# Autodesk Inventor assembly: Chassis Assembly
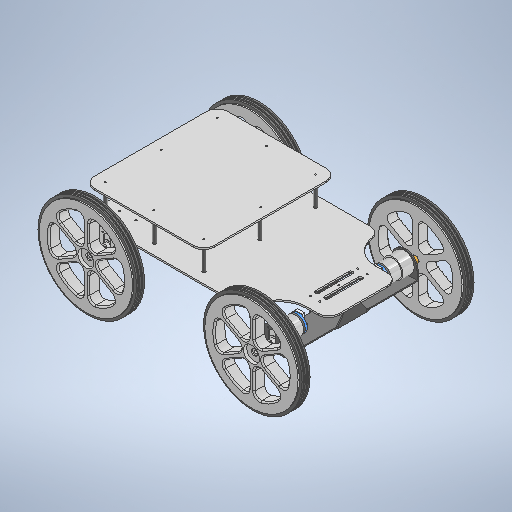
[picture p0: Inventor's stored thumbnail of the model, 512x512]
Saved by Autodesk Inventor 2025.2 (Build 292293000, 293)
## iProperties
Created: 2025-01-16
Part Number: Chassis Assembly
Document SubType Name: Assembly
Designer: Matt Tidd
Author: Matt Tidd
## Documents named in this file (6)
- C:\Users\mtidd2\Desktop\H2A\CAD\Chassis_Design\Chassis Assembly.iam
- C:\Users\mtidd2\Desktop\H2A\CAD\Motors_and_Wheels\Pendulum Suspension\Pendulum Suspension Assembly.iam
- C:\Users\mtidd2\Desktop\H2A\CAD\Chassis_Design\Chassis Bottom Plate.ipt
- C:\Users\mtidd2\Desktop\H2A\CAD\Motors_and_Wheels\Wheel Assembly\Motor Wheel Assembly.iam
- C:\Users\mtidd2\Desktop\H2A\CAD\Chassis_Design\Support Columns.ipt
- C:\Users\mtidd2\Desktop\H2A\CAD\Chassis_Design\Chassis Top Plate.ipt
## Components (13 placed, 5 different names)
1. Pendulum Suspension Assembly:1 [sub-assembly] — Rigid:12
2. Chassis Bottom Plate:1 — Rigid:1, Rigid:2, Rigid:3, Rigid:4, Rigid:5, Rigid:6, Rigid:7, Rigid:8, Rigid:10, Rigid:11, Rigid:12
3. Motor Wheel Assembly:1 [sub-assembly] — Rigid:11
4. Motor Wheel Assembly:2 [sub-assembly] — Rigid:10
5. Chassis Top Plate:1 — Rigid:9
6. Support Columns:1 — Rigid:5
7. Support Columns:2 — Rigid:6
8. Support Columns:3 — Rigid:1
9. Support Columns:4 — Rigid:4
10. Support Columns:5 — Rigid:2, Rigid:9
11. Support Columns:6 — Rigid:7
12. Support Columns:7 — Rigid:8
13. Support Columns:8 — Rigid:3
## Relationships (12: WeldJoint 12)
- Rigid:1 [WeldJoint]: Chassis Bottom Plate:1 ↔ Support Columns:3
- Rigid:2 [WeldJoint]: Chassis Bottom Plate:1 ↔ Support Columns:5
- Rigid:3 [WeldJoint]: Chassis Bottom Plate:1 ↔ Support Columns:8
- Rigid:4 [WeldJoint]: Chassis Bottom Plate:1 ↔ Support Columns:4
- Rigid:5 [WeldJoint]: Chassis Bottom Plate:1 ↔ Support Columns:1
- Rigid:6 [WeldJoint]: Chassis Bottom Plate:1 ↔ Support Columns:2
- Rigid:7 [WeldJoint]: Chassis Bottom Plate:1 ↔ Support Columns:6
- Rigid:8 [WeldJoint]: Chassis Bottom Plate:1 ↔ Support Columns:7
- Rigid:9 [WeldJoint] (50 mm): Chassis Top Plate:1 ↔ Support Columns:5
- Rigid:10 [WeldJoint]: Chassis Bottom Plate:1 ↔ Motor Wheel Assembly:2
- Rigid:11 [WeldJoint]: Chassis Bottom Plate:1 ↔ Motor Wheel Assembly:1
- Rigid:12 [WeldJoint]: Pendulum Suspension Assembly:1 ↔ Chassis Bottom Plate:1
